# Autodesk Inventor assembly: arm assembly
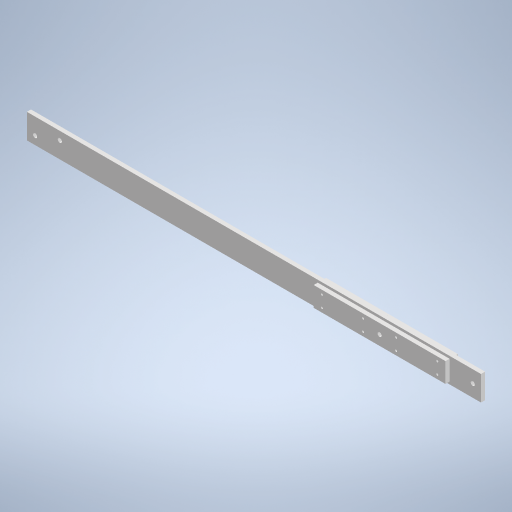
[picture p0: Inventor's stored thumbnail of the model, 512x512]
Saved by Autodesk Inventor 2023 (Build 270158000, 158)
## iProperties
Created: 2023-10-16
Part Number: arm assembly
Document SubType Name: Assembly
Designer: Nate
Author: Nate
## Documents named in this file (4)
- C:\Users\Nate\Desktop\Trebuchet\arm assembly.iam
- C:\Users\Nate\Desktop\Trebuchet\arm counterweight.ipt
- C:\Users\Nate\Desktop\Trebuchet\arm.ipt
- C:\Users\Nate\Desktop\Trebuchet\arm projectile.ipt
## Components (4 placed, 3 different names)
1. arm counterweight:1 — Mate:1, Mate:2
2. arm:1 — Mate:4
3. arm:2 — Mate:3
4. arm projectile:1 — Mate:1, Mate:2, Mate:3, Mate:4
## Relationships (4: Mate 4)
- Mate:1: arm counterweight:1 ↔ arm projectile:1
- Mate:2: arm counterweight:1 ↔ arm projectile:1
- Mate:3: arm:2 ↔ arm projectile:1
- Mate:4: arm:1 ↔ arm projectile:1
